# Autodesk Inventor assembly: MotorSoporte
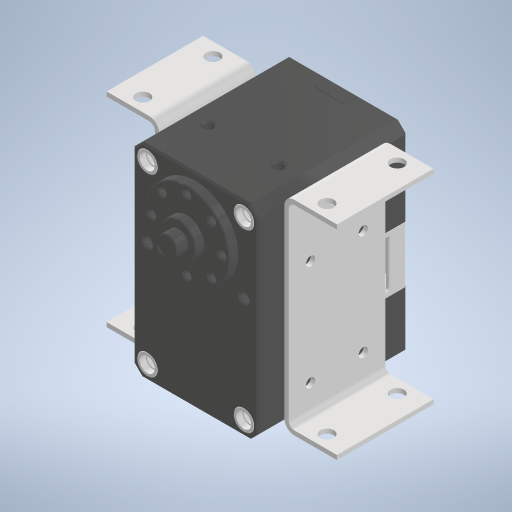
[picture p0: Inventor's stored thumbnail of the model, 512x512]
Saved by Autodesk Inventor 2023.1 (Build 271208000, 208)
## iProperties
Created: 2022-09-08
Part Number: MotorSoporte
Document SubType Name: Assembly
Designer: Lab. de Manufactura
Author: Lab. de Manufactura
## Documents named in this file (3)
- C:\Users\Lab. de Manufactura\Desktop\SSL\Jean\MotorSoporte.iam
- C:\Users\Lab. de Manufactura\Desktop\SSL\Jean\Motor X430_STD\X430_STD.iam
- C:\Users\Lab. de Manufactura\Desktop\SSL\Jean\MotorSoport.ipt
## Components (3 placed, 2 different names)
1. X430_STD:1 [sub-assembly] — Rígido:1, Rígido:2
2. MotorSoport:1 — Rígido:1
3. MotorSoport:2 — Rígido:2
## Relationships (2: WeldJoint 2)
- Rígido:1 [WeldJoint]: X430_STD:1 ↔ MotorSoport:1
- Rígido:2 [WeldJoint]: X430_STD:1 ↔ MotorSoport:2
